# Autodesk Inventor assembly: ArmSolenoidShaft
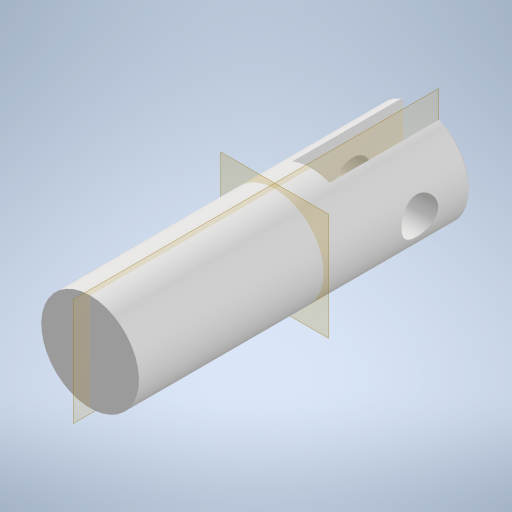
[picture p0: Inventor's stored thumbnail of the model, 512x512]
Saved by Autodesk Inventor 2023 (Build 270158000, 158)
## iProperties
Created: 2023-03-29
Part Number: ArmSolenoidShaft
Document SubType Name: Assembly
Designer: LattePanda
Author: LattePanda
## Documents named in this file (2)
- C:\Users\LattePanda\Desktop\str1ker\description\models\src\ArmSolenoidShaft.iam
- C:\Users\LattePanda\Desktop\str1ker\parts\external\ArmSolenoidShaft.ipt
## Components (1 placed, 1 different names)
1. ArmSolenoidShaft:1 — Mate:1, Flush:1, Angle:1
## Relationships (3: Mate 1, Flush 1, Angle 1)
- Mate:1: ArmSolenoidShaft:1
- Flush:1 (12 mm): ArmSolenoidShaft:1
- Angle:1 (0 deg): ArmSolenoidShaft:1
